# Autodesk Inventor assembly: Single Track 9-24-19
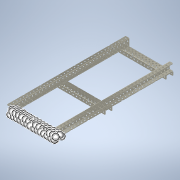
[picture p0: Inventor's stored thumbnail of the model, 180x180]
Saved by Autodesk Inventor 2020 (Build 240168000, 168)
## iProperties
Created: 2019-09-25
Part Number: Single Track 9-24-19
Document SubType Name: Assembly
Designer: spenc
Author: spenc
## Documents named in this file (3)
- C:\Users\spenc\OneDrive\Desktop\Vex Robotics\Tower-Takeover-CAD\Single Track 9-24-19.iam
- C:\Users\spenc\OneDrive\Desktop\Vex Robotics\Tower-Takeover-CAD\Parts\Structure\C-Channels\Aluminum\2-Wide\Aluminum C-Channel 1x2x1x14.ipt
- C:\Users\spenc\OneDrive\Desktop\Vex Robotics\Tower-Takeover-CAD\Parts\Structure\C-Channels\Aluminum\2-Wide\Aluminum C-Channel 1x2x1x35.ipt
## Components (5 placed, 2 different names)
1. Aluminum C-Channel 1x2x1x14:1 — Mate:1, Flush:1, Mate:4
2. Aluminum C-Channel 1x2x1x14:2 — Mate:2, Flush:2
3. Aluminum C-Channel 1x2x1x14:3 — Mate:3, Flush:3
4. Aluminum C-Channel 1x2x1x35:1 — Mate:1, Flush:1, Mate:2, Flush:2, Mate:3, Flush:3
5. Aluminum C-Channel 1x2x1x35:2 — Mate:4
## Relationships (7: Mate 4, Flush 3)
- Mate:1: Aluminum C-Channel 1x2x1x14:1 ↔ Aluminum C-Channel 1x2x1x35:1
- Flush:1: Aluminum C-Channel 1x2x1x14:1 ↔ Aluminum C-Channel 1x2x1x35:1
- Mate:2: Aluminum C-Channel 1x2x1x14:2 ↔ Aluminum C-Channel 1x2x1x35:1
- Flush:2: Aluminum C-Channel 1x2x1x14:2 ↔ Aluminum C-Channel 1x2x1x35:1
- Mate:3: Aluminum C-Channel 1x2x1x14:3 ↔ Aluminum C-Channel 1x2x1x35:1
- Flush:3: Aluminum C-Channel 1x2x1x14:3 ↔ Aluminum C-Channel 1x2x1x35:1
- Mate:4: Aluminum C-Channel 1x2x1x14:1 ↔ Aluminum C-Channel 1x2x1x35:2
